# Autodesk Inventor assembly: V-Belt transmission
Saved by Autodesk Inventor 2014 (Build 180170000, 170)
## iProperties
Created: 2017-06-15
Part Number: V-Belt transmission
Document SubType Name: Assembly
Designer: RMcComber
ClientObjectVersion: 1
Author: RMcComber
## Documents named in this file (4)
- C:\Users\rmccomber\Documents\st motor\electronic valving\2017\engine\Design Accelerator\V-Belt transmission1.iam
- C:\Users\rmccomber\Documents\st motor\electronic valving\2017\engine\Design Accelerator\V-Belt1.ipt
- C:\Users\rmccomber\Documents\st motor\electronic valving\2017\engine\Design Accelerator\Grooved Pulley11.ipt
- C:\Users\rmccomber\Documents\st motor\electronic valving\2017\engine\Design Accelerator\Grooved Pulley21.ipt
## Components (3 placed, 3 different names)
1. Grooved Pulley1:1 — Flush:1, Mate:1, Rotation:1
2. Grooved Pulley2:1 — Flush:2, Mate:2, Rotation:1
3. V-Belt:1 — Flush:1, Mate:1, Flush:2, Mate:2
## Component patterns: (1 elements, first: V-Belt:1)
## Relationships (5: Flush 2, Mate 2, RelateRotation 1)
- Flush:1: Grooved Pulley1:1 ↔ V-Belt:1
- Mate:1: Grooved Pulley1:1 ↔ V-Belt:1
- Flush:2: Grooved Pulley2:1 ↔ V-Belt:1
- Mate:2: Grooved Pulley2:1 ↔ V-Belt:1
- Rotation:1 [RelateRotation] (1 ul): Grooved Pulley1:1 ↔ Grooved Pulley2:1
